# Autodesk Inventor assembly: !Hook
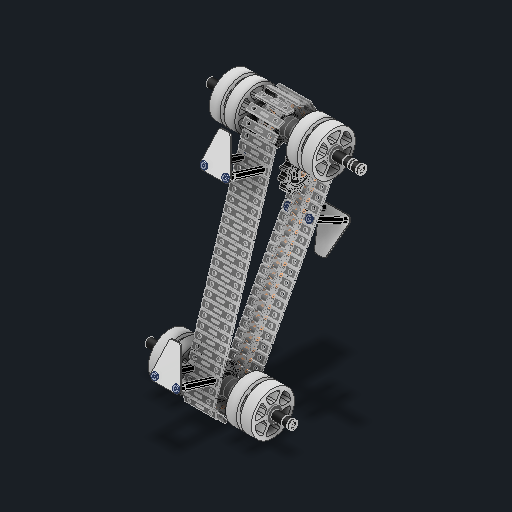
[picture p0: Inventor's stored thumbnail of the model, 512x512]
Saved by Autodesk Inventor 2025.1 (Build 291241000, 241)
## iProperties
Created: 2024-10-20
Part Number: !Hook
Document SubType Name: Assembly
Designer: Averey Ku
Author: Averey Ku
## Documents named in this file (11)
- C:\Users\avere\VEX\High Stakes\CAD\V2\Hook\!Hook.iam
- C:\Users\avere\VEX\High Stakes\CAD\V2\Hook\Chain.iam
- C:\Users\avere\VEX\High Stakes\CAD\ROBOPROS-CAD-Inventor\Structure\Hardware\Screw Shoulder Robosource\SScrew Shoulder Smooth .500 x .04.ipt
- C:\Users\avere\VEX\High Stakes\CAD\ROBOPROS-CAD-Inventor\Motion\Sprockets\9P Sprocket\9P 12T Sprocket, No Insert.iam
- C:\Users\avere\VEX\High Stakes\CAD\V2\Hook\Roller Shaft.iam
- C:\Users\avere\VEX\High Stakes\CAD\ROBOPROS-CAD-Inventor\Structure\Hardware\Screw Shoulder Robosource.ipt
- C:\Users\avere\VEX\High Stakes\CAD\ROBOPROS-CAD-Inventor\Motion\Sprockets\9P Sprocket.iam
- C:\Users\avere\VEX\High Stakes\CAD\ROBOPROS-CAD-Inventor\Motion\Shaft HS\HS Spacer\HSpacer .1250.ipt
- C:\Users\avere\VEX\High Stakes\CAD\ROBOPROS-CAD-Inventor\Motion\Shaft HS\HS Spacer.ipt
- C:\Users\avere\VEX\High Stakes\CAD\ROBOPROS-CAD-Inventor\Motion\Shaft HS\HS Spacer\HSpacer .2500.ipt
- C:\Users\avere\VEX\High Stakes\CAD\V2\Hook\Individual Hook.iam
## Components (19 placed, 7 different names)
1. Chain:1 [sub-assembly] — Insert:9, Insert:10, Mate:9, Insert:37, Mate:13, Insert:41, Mate:14, Insert:42, Insert:43, Insert:44, Mate:15
2. Roller Shaft:1 [sub-assembly] — Flush:1, Mate:10
3. Roller Shaft:2 [sub-assembly] — Flush:2, Insert:33, Insert:35
4. 9P 12T Sprocket, No Insert:1 [sub-assembly] — Mate:9, Mate:10
5. HSpacer .1250:1 — Insert:32
6. HSpacer .2500:2 — Insert:32, Insert:33
7. HSpacer .1250:3
8. HSpacer .2500:4 — Insert:35
9. SScrew Shoulder Smooth .500 x .04:17
10. SScrew Shoulder Smooth .500 x .04:18
11. Individual Hook:1 [sub-assembly] — Insert:42, Insert:43
12. Individual Hook:2 [sub-assembly] — Insert:41, Mate:14
13. Individual Hook:3 [sub-assembly] — Mate:13, Insert:44, Mate:15
14. SScrew Shoulder Smooth .500 x .04:3 — Insert:10
15. SScrew Shoulder Smooth .500 x .04:4 — Insert:9
16. SScrew Shoulder Smooth .500 x .04:8 — Insert:37
17. SScrew Shoulder Smooth .500 x .04:7
18. SScrew Shoulder Smooth .500 x .04:11
19. SScrew Shoulder Smooth .500 x .04:12
## Relationships (18: Insert 11, Mate 5, Flush 2)
- Insert:9: Chain:1 ↔ SScrew Shoulder Smooth .500 x .04:4
- Insert:10: Chain:1 ↔ SScrew Shoulder Smooth .500 x .04:3
- Flush:1 (6.35 mm): Roller Shaft:1
- Flush:2 (6.35 mm): Roller Shaft:2
- Mate:9: Chain:1 ↔ 9P 12T Sprocket, No Insert:1
- Mate:10: Roller Shaft:1 ↔ 9P 12T Sprocket, No Insert:1
- Insert:32: HSpacer .1250:1 ↔ HSpacer .2500:2
- Insert:33: Roller Shaft:2 ↔ HSpacer .2500:2
- [Insert]: HSpacer .1250:3 ↔ HSpacer .2500:4
- Insert:35: Roller Shaft:2 ↔ HSpacer .2500:4
- Insert:37: Chain:1 ↔ SScrew Shoulder Smooth .500 x .04:8
- Mate:13: Chain:1 ↔ Individual Hook:3
- Insert:41: Chain:1 ↔ Individual Hook:2
- Mate:14: Chain:1 ↔ Individual Hook:2
- Insert:42: Chain:1 ↔ Individual Hook:1
- Insert:43: Chain:1 ↔ Individual Hook:1
- Insert:44: Chain:1 ↔ Individual Hook:3
- Mate:15: Chain:1 ↔ Individual Hook:3
## Named parameters: d73_d71 = 0 mm
